# Autodesk Inventor assembly: conj-mao
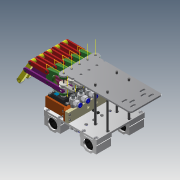
[picture p0: Inventor's stored thumbnail of the model, 180x180]
Saved by Autodesk Inventor 2017 (Build 210142000, 142)
## iProperties
Created: 2018-06-16
Part Number: conj-mao
Document SubType Name: Assembly
Designer: Luiz Gustavo
Author: Luiz Gustavo
## Documents named in this file (16)
- C:\Users\Luiz Gustavo\Documents\Inventor\piano-robot\conj-mao.iam
- C:\Users\Luiz Gustavo\Documents\Inventor\piano-robot\servo-holder-1.ipt
- C:\Users\Luiz Gustavo\Documents\Inventor\piano-robot\finger-assembly.iam
- C:\Users\Luiz Gustavo\Documents\Inventor\piano-robot\top-plate.ipt
- C:\Users\Luiz Gustavo\Documents\Inventor\piano-robot\cylinder-holder-1.ipt
- C:\Users\Luiz Gustavo\Documents\Inventor\piano-robot\bottom-plate.ipt
- C:\Users\Luiz Gustavo\Documents\Inventor\piano-robot\grabcad\cs16uu-1.snapshot.1\SC16.ipt
- C:\Users\Luiz Gustavo\Documents\Inventor\piano-robot\fixador-correia.ipt
- C:\Users\Luiz Gustavo\Documents\Inventor\piano-robot\conj-mao\Design Accelerator\Bolted Connection5.iam
- C:\Users\Luiz Gustavo\Documents\Inventor\piano-robot\barra-roscada.ipt
- C:\Users\Luiz Gustavo\Documents\Inventor\piano-robot\conj-mao\Design Accelerator\Bolted Connection1.iam
- C:\Users\Luiz Gustavo\Documents\Inventor\piano-robot\conj-mao\Design Accelerator\Bolted Connection2.iam
- C:\Users\Luiz Gustavo\Documents\Inventor\piano-robot\conj-mao\Design Accelerator\Bolted Connection3.iam
- C:\Users\Luiz Gustavo\Documents\Inventor\piano-robot\conj-mao\Design Accelerator\Bolted Connection4.iam
- C:\Users\Luiz Gustavo\Documents\Inventor\piano-robot\agregador-cilindros.ipt
- C:\Users\Luiz Gustavo\Documents\Inventor\piano-robot\conj-mao\Design Accelerator\Bolted Connection6.iam
## Components (26 placed, 10 different names)
1. servo-holder-1:1 — Mate:1, Mate:2, Mate:3, Mate:4, Mate:5, Mate:6, Flush:1, Flush:2, Flush:3, Mate:7, Mate:8, Mate:9, Mate:10, Mate:11, Mate:12, Mate:13, Mate:14, Mate:15, Flush:5, Flush:6
2. finger-assembly:1 [sub-assembly] — Mate:1, Mate:2, Mate:3, Mate:17, Mate:46, Mate:47
3. finger-assembly:2 [sub-assembly] — Mate:4, Mate:5, Mate:6
4. finger-assembly:3 [sub-assembly] — Mate:7, Mate:8, Mate:9, Mate:19, Rigid:11
5. finger-assembly:4 [sub-assembly] — Mate:13, Mate:14, Mate:15, Mate:18, Mate:36, Mate:37
6. finger-assembly:5 [sub-assembly] — Mate:10, Mate:11, Mate:12
7. top-plate:1 — Mate:17, Mate:18, Mate:19, Mate:48, Mate:49
8. cylinder-holder-1:1 — Flush:5, Mate:32, Mate:33
9. bottom-plate:1 — Flush:6, Rigid:1, Rigid:2, Rigid:3, Rigid:4, Rigid:5, Rigid:6, Rigid:7, Rigid:10, Rigid:8, Rigid:9, Mate:34, Mate:35
10. SC16:1 — Rigid:1
11. SC16:2 — Rigid:2
12. SC16:3 — Rigid:4
13. SC16:4 — Rigid:3
14. fixador-correia:1 — Rigid:5
15. fixador-correia:2 — Rigid:6, Mate:40, Mate:41
16. Bolted Connection:1 [sub-assembly] — Mate:32, Mate:33
17. barra-roscada:1 — Rigid:7
18. barra-roscada:2 — Rigid:9
19. barra-roscada:3 — Rigid:8
20. barra-roscada:4 — Rigid:10
21. Bolted Connection:2 [sub-assembly] — Mate:34, Mate:35
22. Bolted Connection:3 [sub-assembly] — Mate:40, Mate:41
23. Bolted Connection:4 [sub-assembly] — Mate:36, Mate:37
24. Bolted Connection:5 [sub-assembly] — Mate:48, Mate:49
25. agregador-cilindros:1 — Rigid:11
26. Bolted Connection:6 [sub-assembly] — Mate:46, Mate:47
## Relationships (46: Mate 30, WeldJoint 11, Flush 5)
- Mate:1: servo-holder-1:1 ↔ finger-assembly:1
- Mate:2: servo-holder-1:1 ↔ finger-assembly:1
- Mate:3: servo-holder-1:1 ↔ finger-assembly:1
- Mate:4: servo-holder-1:1 ↔ finger-assembly:2
- Mate:5: servo-holder-1:1 ↔ finger-assembly:2
- Mate:6: servo-holder-1:1 ↔ finger-assembly:2
- Flush:1: servo-holder-1:1
- Flush:2: servo-holder-1:1
- Flush:3: servo-holder-1:1
- Mate:7: servo-holder-1:1 ↔ finger-assembly:3
- Mate:8: servo-holder-1:1 ↔ finger-assembly:3
- Mate:9: servo-holder-1:1 ↔ finger-assembly:3
- Mate:10: servo-holder-1:1 ↔ finger-assembly:5
- Mate:11: servo-holder-1:1 ↔ finger-assembly:5
- Mate:12: servo-holder-1:1 ↔ finger-assembly:5
- Mate:13: servo-holder-1:1 ↔ finger-assembly:4
- Mate:14: servo-holder-1:1 ↔ finger-assembly:4
- Mate:15: servo-holder-1:1 ↔ finger-assembly:4
- Mate:17: finger-assembly:1 ↔ top-plate:1
- Mate:18: finger-assembly:4 ↔ top-plate:1
- Mate:19: finger-assembly:3 ↔ top-plate:1
- Flush:5: servo-holder-1:1 ↔ cylinder-holder-1:1
- Flush:6: servo-holder-1:1 ↔ bottom-plate:1
- Rigid:1 [WeldJoint]: bottom-plate:1 ↔ SC16:1
- Rigid:2 [WeldJoint]: bottom-plate:1 ↔ SC16:2
- Rigid:3 [WeldJoint]: bottom-plate:1 ↔ SC16:4
- Rigid:4 [WeldJoint]: bottom-plate:1 ↔ SC16:3
- Rigid:5 [WeldJoint] (-3 mm): bottom-plate:1 ↔ fixador-correia:1
- Rigid:6 [WeldJoint] (-3 mm): bottom-plate:1 ↔ fixador-correia:2
- Rigid:7 [WeldJoint] (15 mm): bottom-plate:1 ↔ barra-roscada:1
- Rigid:10 [WeldJoint] (15 mm): bottom-plate:1 ↔ barra-roscada:4
- Rigid:8 [WeldJoint] (15 mm): bottom-plate:1 ↔ barra-roscada:3
- Rigid:9 [WeldJoint] (15 mm): bottom-plate:1 ↔ barra-roscada:2
- Mate:32: cylinder-holder-1:1 ↔ Bolted Connection:1
- Mate:33: cylinder-holder-1:1 ↔ Bolted Connection:1
- Mate:34: bottom-plate:1 ↔ Bolted Connection:2
- Mate:35: bottom-plate:1 ↔ Bolted Connection:2
- Mate:36: finger-assembly:4 ↔ Bolted Connection:4
- Mate:37: finger-assembly:4 ↔ Bolted Connection:4
- Mate:40: fixador-correia:2 ↔ Bolted Connection:3
- Mate:41: fixador-correia:2 ↔ Bolted Connection:3
- Rigid:11 [WeldJoint]: finger-assembly:3 ↔ agregador-cilindros:1
- Mate:46: finger-assembly:1 ↔ Bolted Connection:6
- Mate:47: finger-assembly:1 ↔ Bolted Connection:6
- Mate:48: top-plate:1 ↔ Bolted Connection:5
- Mate:49: top-plate:1 ↔ Bolted Connection:5
